# Autodesk Inventor assembly: Assembly suelo
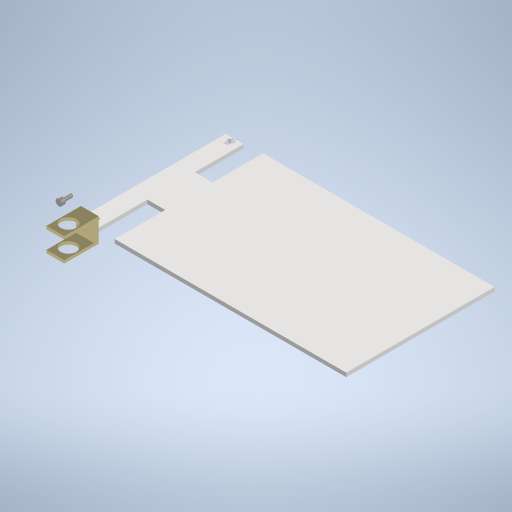
[picture p0: Inventor's stored thumbnail of the model, 512x512]
Saved by Autodesk Inventor 2024 (Build 280153000, 153)
## iProperties
Created: 2023-05-06
Part Number: Assembly suelo
Document SubType Name: Assembly
Designer: Diego
Author: Diego
## Documents named in this file (4)
- C:\Users\Diego\Desktop\Proyecto2_micros\Assembly suelo.iam
- C:\Users\Diego\Desktop\Proyecto2_micros\suelo_imp.ipt
- C:\Users\Diego\Desktop\Proyecto2_micros\tornillo_5_5_10_5.ipt
- C:\Users\Diego\Desktop\Proyecto2_micros\llanta_1.ipt
## Components (3 placed, 3 different names)
1. suelo_imp:1 — Rigid:1
2. tornillo_5_5_10_5:1
3. llanta_1:1 — Rigid:1
## Relationships (1: WeldJoint 1)
- Rigid:1 [WeldJoint] (7.5 mm): suelo_imp:1 ↔ llanta_1:1
